# Autodesk Inventor assembly: 217-2 Stage Versaplanetary STEP
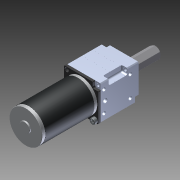
[picture p0: Inventor's stored thumbnail of the model, 180x180]
Saved by Autodesk Inventor 2014 SP1 (Build 180222100, 222)
## iProperties
Created: 2014-01-06
Part Number: 217-2 Stage Versaplanetary STEP
Document SubType Name: Assembly
Designer: Arpan
Mass: 257.085 g
Surface Area: 545.557 cm^2
Volume: 154.963 cm^3
Density: 1.65901 g/cm^3
Title: 217-2 Stage Versaplanetary STEP.STEP
Description: STEP AP214
Creation Date: 2013-12-10
Sending System: SolidWorks 2013
Preprocessor: SwSTEP 2.0
Author: Arpan
## Documents named in this file (14)
- C:\Users\Arpan\Documents\GitHub\2014buildCAD\Shooter\Shooter v1 (Defunct)\217-2 Stage Versaplanetary STEP.iam
- C:\Users\Arpan\Documents\GitHub\2014buildCAD\Imported Components\217-2 Stage Versaplanetary STEP\217-2625-001 Rev1.ipt
- C:\Users\Arpan\Documents\GitHub\2014buildCAD\Imported Components\217-2 Stage Versaplanetary STEP\217-2625-002 Rev1.ipt
- C:\Users\Arpan\Documents\GitHub\2014buildCAD\Imported Components\217-2 Stage Versaplanetary STEP\217-2625-009 Rev1.ipt
- C:\Users\Arpan\Documents\GitHub\2014buildCAD\Imported Components\217-2 Stage Versaplanetary STEP\217-2816-001 Rev1.ipt
- C:\Users\Arpan\Documents\GitHub\2014buildCAD\Imported Components\217-2 Stage Versaplanetary STEP\217-2625-007 Rev1_Sun_Driver01.ipt
- C:\Users\Arpan\Documents\GitHub\2014buildCAD\Imported Components\217-2 Stage Versaplanetary STEP\217-2625-100.iam
- C:\Users\Arpan\Documents\GitHub\2014buildCAD\Imported Components\217-2 Stage Versaplanetary STEP\217-2822-003 Rev4.ipt
- C:\Users\Arpan\Documents\GitHub\2014buildCAD\Imported Components\217-2 Stage Versaplanetary STEP\217-2625-011 Rev1.ipt
- C:\Users\Arpan\Documents\GitHub\2014buildCAD\Imported Components\217-2 Stage Versaplanetary STEP\SSA_SSA0832-0500ZC.ipt
- C:\Users\Arpan\Documents\GitHub\2014buildCAD\Imported Components\217-2 Stage Versaplanetary STEP\217-2742.ipt
- C:\Users\Arpan\Documents\GitHub\2014buildCAD\Imported Components\217-2 Stage Versaplanetary STEP\PINL-M020-006-S.ipt
- C:\Users\Arpan\Documents\GitHub\2014buildCAD\Imported Components\217-2 Stage Versaplanetary STEP\217-3351.ipt
- C:\Users\Arpan\Documents\GitHub\2014buildCAD\Shooter\Shooter v1 (Defunct)\Vex Pro 0.500 Hex VersaPlanetary Output.ipt
## Components (14 placed, 14 different names)
1. 217-2625-001 Rev1_1
2. 217-2625-009 Rev1_4
3. 217-2816-001 Rev1_5 — Mate:1, Flush:1, Flush:2
4. 217-2625-007 Rev1_Sun_Driver01_6
5. 217-2625-100_7 [sub-assembly]
6. 217-2822-003 Rev4_8
7. 217-2625-011 Rev1_9
8. SSA_SSA0832-0500ZC_10
9. PINL-M020-006-S_17
10. PINL-M020-006-S_18
11. 217-3351_19
12. 217-2742_12 — Insert:1, Insert:2
13. 217-2625-002 Rev1_2 — Mate:1, Flush:1, Flush:2, Insert:1
14. Vex Pro 0.500 Hex VersaPlanetary Output:1 — Insert:2
## Relationships (5: Flush 2, Insert 2, Mate 1)
- Mate:1: 217-2816-001 Rev1_5 ↔ 217-2625-002 Rev1_2
- Flush:1: 217-2816-001 Rev1_5 ↔ 217-2625-002 Rev1_2
- Flush:2: 217-2816-001 Rev1_5 ↔ 217-2625-002 Rev1_2
- Insert:1: 217-2742_12 ↔ 217-2625-002 Rev1_2
- Insert:2: 217-2742_12 ↔ Vex Pro 0.500 Hex VersaPlanetary Output:1
